# Autodesk Inventor assembly: Robot
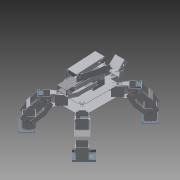
[picture p0: Inventor's stored thumbnail of the model, 180x180]
Saved by Autodesk Inventor 2013 (Build 170138000, 138)
## iProperties
Created: 2014-04-09
Part Number: Robot
Document SubType Name: Assembly
Designer: andou
Author: andou
## Documents named in this file (5)
- C:\Users\andou\Documents\GitHub\Robotics-Project\design\RoboticsProject\project_4\Robot.iam
- C:\Users\andou\Documents\GitHub\Robotics-Project\design\RoboticsProject\project_4\Body.iam
- C:\Users\andou\Documents\GitHub\Robotics-Project\design\RoboticsProject\project_4\Arm.iam
- C:\Users\andou\Documents\GitHub\Robotics-Project\design\RoboticsProject\project_4\Generic Parts\Low_Height_Horn.ipt
- C:\Users\andou\Documents\GitHub\Robotics-Project\design\RoboticsProject\project_4\Generic Parts\KRS-2542HV.ipt
## Components (4 placed, 4 different names)
1. Body:1 [sub-assembly] — 挿入:1, 挿入:2
2. Arm:1 [sub-assembly] — 挿入:4, 挿入:5
3. Low_Height_Horn:1 — 挿入:3, 挿入:4, 挿入:5
4. KRS-2542HV:1 — 挿入:1, 挿入:2, 挿入:3
## Relationships (5: Insert 5)
- 挿入:1 [Insert]: Body:1 ↔ KRS-2542HV:1
- 挿入:2 [Insert]: Body:1 ↔ KRS-2542HV:1
- 挿入:3 [Insert]: Low_Height_Horn:1 ↔ KRS-2542HV:1
- 挿入:4 [Insert]: Arm:1 ↔ Low_Height_Horn:1
- 挿入:5 [Insert]: Arm:1 ↔ Low_Height_Horn:1
